# Autodesk Inventor assembly: Robot Triciclo - Ensamble
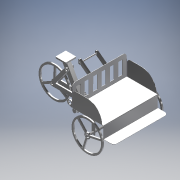
[picture p0: Inventor's stored thumbnail of the model, 180x180]
Saved by Autodesk Inventor 2019 (Build 230136000, 136)
## iProperties
Created: 2019-11-14
Part Number: Robot Triciclo - Ensamble
Document SubType Name: Weldment
Designer: eddysanoli
Weld Material: Welded Aluminum-6061
Author: eddysanoli
## Documents named in this file (7)
- E:\Archivos\Diseño\Inventor\Diseño Mecánico II\Proyecto - Hombre en Bicicleta\Mecanismos_Diseno\Robot Triciclo - Ensamble.iam
- E:\Archivos\Diseño\Inventor\Diseño Mecánico II\Proyecto - Hombre en Bicicleta\Mecanismos_Diseno\Asiento - Ensamble.iam
- E:\Archivos\Diseño\Inventor\Diseño Mecánico II\Proyecto - Hombre en Bicicleta\Mecanismos_Diseno\Marco_triciclo.iam
- E:\Archivos\Diseño\Inventor\Diseño Mecánico II\Proyecto - Hombre en Bicicleta\Mecanismos_Diseno\Rueda_triciclo.ipt
- E:\Archivos\Diseño\Inventor\Diseño Mecánico II\Proyecto - Hombre en Bicicleta\Mecanismos_Diseno\Pedal.ipt
- E:\Archivos\Diseño\Inventor\Diseño Mecánico II\Proyecto - Hombre en Bicicleta\Mecanismos_Diseno\Robot Triciclo - Ensamble\Design Accelerator\Eje1.iam
- E:\Archivos\Diseño\Inventor\Diseño Mecánico II\Proyecto - Hombre en Bicicleta\Mecanismos_Diseno\Marco - Asiento Triciclo.ipt
## Components (8 placed, 6 different names)
1. Asiento - Ensamble:1 [sub-assembly] — Coincidencia:1, Coincidencia:2, Nivelación:1, Coincidencia:3, Coincidencia:4, Coincidencia:5, Coincidencia:6, Coincidencia:10
2. Marco_triciclo:2 [sub-assembly] — Coincidencia:1, Coincidencia:2, Nivelación:1, Coincidencia:7, Coincidencia:8, Coincidencia:9, Coincidencia:11, Nivelación:4, Nivelación:5
3. Rueda_triciclo:1 — Coincidencia:3, Coincidencia:5
4. Rueda_triciclo:2 — Coincidencia:4, Coincidencia:6, Nivelación:3
5. Pedal:1 — Nivelación:2, Coincidencia:7, Coincidencia:9
6. Pedal:2 — Nivelación:2, Coincidencia:8
7. Eje:1 [sub-assembly] — Coincidencia:10, Nivelación:3
8. Marco - Asiento Triciclo:1 — Coincidencia:11, Nivelación:4, Nivelación:5
## Relationships (16: Mate 11, Flush 5)
- Coincidencia:1 [Mate]: Asiento - Ensamble:1 ↔ Marco_triciclo:2
- Coincidencia:2 [Mate] (59.8 mm): Asiento - Ensamble:1 ↔ Marco_triciclo:2
- Nivelación:1 [Flush] (183.5 mm): Asiento - Ensamble:1 ↔ Marco_triciclo:2
- Coincidencia:3 [Mate]: Asiento - Ensamble:1 ↔ Rueda_triciclo:1
- Coincidencia:4 [Mate]: Asiento - Ensamble:1 ↔ Rueda_triciclo:2
- Coincidencia:5 [Mate] (35 mm): Asiento - Ensamble:1 ↔ Rueda_triciclo:1
- Coincidencia:6 [Mate] (35 mm): Asiento - Ensamble:1 ↔ Rueda_triciclo:2
- Nivelación:2 [Flush]: Pedal:1 ↔ Pedal:2
- Coincidencia:7 [Mate]: Marco_triciclo:2 ↔ Pedal:1
- Coincidencia:8 [Mate]: Marco_triciclo:2 ↔ Pedal:2
- Coincidencia:9 [Mate]: Marco_triciclo:2 ↔ Pedal:1
- Coincidencia:10 [Mate]: Asiento - Ensamble:1 ↔ Eje:1
- Nivelación:3 [Flush] (-2.5 mm): Rueda_triciclo:2 ↔ Eje:1
- Coincidencia:11 [Mate]: Marco_triciclo:2 ↔ Marco - Asiento Triciclo:1
- Nivelación:4 [Flush] (24 mm): Marco_triciclo:2 ↔ Marco - Asiento Triciclo:1
- Nivelación:5 [Flush] (-20 mm): Marco_triciclo:2 ↔ Marco - Asiento Triciclo:1
